# Autodesk Inventor assembly: Test Lamelo Box
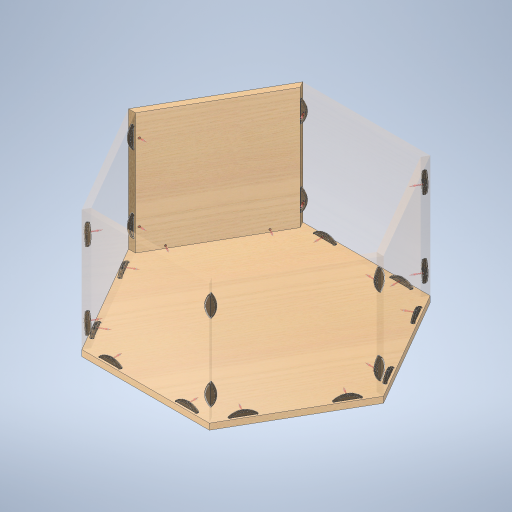
[picture p0: Inventor's stored thumbnail of the model, 512x512]
Saved by Autodesk Inventor 2024 (Build 280153000, 153)
## iProperties
Created: 2021-09-15
Part Number: Test Lamelo Box
Document SubType Name: Assembly
Designer: sauliusd
Author: sauliusd
## Documents named in this file (9)
- C:\W4INV 2024 Design\PROJECTS\Samples\Macro DEMO\5 Lamello Clamex P-14\ClamexTest Box\Test Lamelo Box.iam
- C:\W4INV 2024 Design\PROJECTS\Samples\Macro DEMO\5 Lamello Clamex P-14\ClamexTest Box\Side 1.ipt
- C:\W4INV 2024 Design\PROJECTS\Samples\Macro DEMO\5 Lamello Clamex P-14\ClamexTest Box\Side 2.ipt
- C:\W4INV 2024 Design\PROJECTS\Samples\Macro DEMO\5 Lamello Clamex P-14\ClamexTest Box\Side 3.ipt
- C:\W4INV 2024 Design\PROJECTS\Samples\Macro DEMO\5 Lamello Clamex P-14\ClamexTest Box\Side 4.ipt
- C:\W4INV 2024 Design\PROJECTS\Samples\Macro DEMO\5 Lamello Clamex P-14\ClamexTest Box\Side 5.ipt
- C:\W4INV 2024 Design\PROJECTS\Samples\Macro DEMO\5 Lamello Clamex P-14\ClamexTest Box\Side 6.ipt
- C:\W4INV 2024 Design\PROJECTS\Samples\Macro DEMO\5 Lamello Clamex P-14\ClamexTest Box\Botom.ipt
- C:\W4INV 2024 Design\PROJECTS\Samples\Macro DEMO\5 Lamello Clamex P-14\Clamex P-14 Connector.iam
## Components (31 placed, 8 different names)
1. Side 1:1
2. Side 2:1 — Edge or Inner Plane:1, Joining Plane Solution 1:1, Joining Plane Solution 1:2, Edge or Inner Plane:2, Joining Plane Solution 1:5, Edge or Inner Plane:5, Joining Plane Solution 1:6, Edge or Inner Plane:6
3. Side 3:1
4. Side 4:1
5. Side 5:1
6. Side 6:1 — Flush:1, Flush:2
7. Botom:1 — Mate:1, Angle:1, Mate:2, Angle:2, Center Point Match Plane:6
8. Clamex P-14 Connector:11 [sub-assembly] — Joining Plane Solution 1:5, Edge or Inner Plane:5, Center Point Match Plane:5
9. Clamex P-14 Connector:12 [sub-assembly] — Joining Plane Solution 1:6, Edge or Inner Plane:6, Center Point Match Plane:6
10. Clamex P-14 Connector:8 [sub-assembly] — Joining Plane Solution 1:2, Edge or Inner Plane:2, Center Point Match Plane:2
11. Clamex P-14 Connector:7 [sub-assembly] — Edge or Inner Plane:1, Center Point Match Plane:1, Transverse orientation plane Solution 2:1, Joining Plane Solution 1:1
12. Clamex P-14 Connector:13 [sub-assembly]
13. Clamex P-14 Connector:14 [sub-assembly]
14. Clamex P-14 Connector:15 [sub-assembly]
15. Clamex P-14 Connector:16 [sub-assembly]
16. Clamex P-14 Connector:17 [sub-assembly]
17. Clamex P-14 Connector:18 [sub-assembly]
18. Clamex P-14 Connector:19 [sub-assembly]
19. Clamex P-14 Connector:20 [sub-assembly]
20. Clamex P-14 Connector:21 [sub-assembly]
21. Clamex P-14 Connector:22 [sub-assembly]
22. Clamex P-14 Connector:23 [sub-assembly]
23. Clamex P-14 Connector:24 [sub-assembly]
24. Clamex P-14 Connector:25 [sub-assembly]
25. Clamex P-14 Connector:26 [sub-assembly]
26. Clamex P-14 Connector:27 [sub-assembly]
27. Clamex P-14 Connector:28 [sub-assembly]
28. Clamex P-14 Connector:29 [sub-assembly]
29. Clamex P-14 Connector:30 [sub-assembly]
30. Clamex P-14 Connector:31 [sub-assembly]
31. Clamex P-14 Connector:32 [sub-assembly]
## Component patterns: (6 elements, first: Clamex P-14 Connector:11 + Clamex P-14 Connector:12 + Clamex P-14 Connector:8 + Clamex P-14 Connector:7)
## Relationships (20: Mate 10, Flush 7, Angle 3)
- Flush:1 (-70 mm): Side 6:1
- Flush:2 (-70 mm): Side 6:1
- Mate:1: Botom:1
- Angle:1 (0 deg): Botom:1
- Flush:3 (80 mm)
- Mate:2: Botom:1
- Angle:2 (0 deg): Botom:1
- Edge or Inner Plane:1 [Mate]: Side 2:1 ↔ Clamex P-14 Connector:7
- Center Point Match Plane:1 [Mate]: Clamex P-14 Connector:7
- Transverse orientation plane Solution 2:1 [Angle] (180 deg): Clamex P-14 Connector:7
- Joining Plane Solution 1:1 [Flush]: Side 2:1 ↔ Clamex P-14 Connector:7
- Joining Plane Solution 1:2 [Flush]: Side 2:1 ↔ Clamex P-14 Connector:8
- Edge or Inner Plane:2 [Mate]: Side 2:1 ↔ Clamex P-14 Connector:8
- Center Point Match Plane:2 [Mate]: Clamex P-14 Connector:8
- Joining Plane Solution 1:5 [Flush]: Side 2:1 ↔ Clamex P-14 Connector:11
- Edge or Inner Plane:5 [Mate]: Side 2:1 ↔ Clamex P-14 Connector:11
- Center Point Match Plane:5 [Mate]: Clamex P-14 Connector:11
- Joining Plane Solution 1:6 [Flush]: Side 2:1 ↔ Clamex P-14 Connector:12
- Edge or Inner Plane:6 [Mate]: Side 2:1 ↔ Clamex P-14 Connector:12
- Center Point Match Plane:6 [Mate]: Botom:1 ↔ Clamex P-14 Connector:12
